# Autodesk Inventor assembly: Assembly1
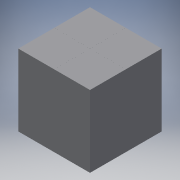
[picture p0: Inventor's stored thumbnail of the model, 180x180]
Saved by Autodesk Inventor 2018 (Build 220112000, 112)
## iProperties
Created: 2020-01-09
Part Number: Assembly1
Document SubType Name: Assembly
Designer: AOFUser
Author: AOFUser
## Documents named in this file (2)
- C:\Users\AOFUser\Desktop\Park_CAD\Assembly1.iam
- C:\Users\AOFUser\Desktop\Park_CAD\cube.ipt
## Components (8 placed, 1 different names)
1. cube:1 — Mate:1, Flush:1, Flush:2, Mate:2, Flush:3, Flush:4, Mate:4, Flush:7, Flush:8
2. cube:2 — Mate:1, Flush:1, Flush:2, Mate:7, Flush:13
3. cube:3 — Mate:3, Flush:5, Flush:6, Mate:6, Flush:12
4. cube:4 — Mate:2, Flush:3, Flush:4, Mate:3, Flush:5, Flush:6, Mate:5, Flush:10
5. cube:5 — Mate:5, Flush:9, Flush:10, Flush:11
6. cube:6 — Mate:6, Flush:11, Flush:12
7. cube:7 — Mate:7, Flush:13, Flush:14
8. cube:8 — Mate:4, Flush:7, Flush:8, Flush:9, Flush:14
## Relationships (21: Flush 14, Mate 7)
- Mate:1: cube:1 ↔ cube:2
- Flush:1: cube:1 ↔ cube:2
- Flush:2: cube:1 ↔ cube:2
- Mate:2: cube:1 ↔ cube:4
- Flush:3: cube:1 ↔ cube:4
- Flush:4: cube:1 ↔ cube:4
- Mate:3: cube:3 ↔ cube:4
- Flush:5: cube:3 ↔ cube:4
- Flush:6: cube:3 ↔ cube:4
- Mate:4: cube:1 ↔ cube:8
- Flush:7: cube:1 ↔ cube:8
- Flush:8: cube:1 ↔ cube:8
- Mate:5: cube:4 ↔ cube:5
- Flush:9: cube:5 ↔ cube:8
- Flush:10: cube:4 ↔ cube:5
- Mate:6: cube:3 ↔ cube:6
- Flush:11: cube:5 ↔ cube:6
- Flush:12: cube:3 ↔ cube:6
- Mate:7: cube:2 ↔ cube:7
- Flush:13: cube:2 ↔ cube:7
- Flush:14: cube:7 ↔ cube:8
